# Autodesk Inventor assembly: Сборка1
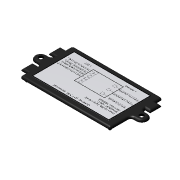
[picture p0: Inventor's stored thumbnail of the model, 180x180]
Saved by Autodesk Inventor 2012 (Build 160160000, 160)
## iProperties
Created: 2009-10-05
Part Number: Сборка1
Document SubType Name: Assembly
Designer: toma
Mass: 4.81656 g
Surface Area: 92.9962 cm^2
Volume: 4.81656 cm^3
Density: 1 g/cm^3
Author: toma
## Documents named in this file (3)
- D:\VSS_WORK\VSS_ENERGO\Сумматор light\КД\Сумматор Light\Сборка1.iam
- D:\VSS_WORK\VSS_ENERGO\Сумматор light\КД\Сумматор Light\крышка.ipt
- D:\VSS_WORK\VSS_ENERGO\Сумматор light\КД\Сумматор Light\наклейка.ipt
## Components (2 placed, 2 different names)
1. крышка:1 — Совмещение:1, Совмещение:2, Совмещение:3
2. наклейка:1 — Совмещение:1, Совмещение:2, Совмещение:3
## Relationships (3: Mate 3)
- Совмещение:1 [Mate]: крышка:1 ↔ наклейка:1
- Совмещение:2 [Mate] (3.5 mm): крышка:1 ↔ наклейка:1
- Совмещение:3 [Mate] (2.5 mm): крышка:1 ↔ наклейка:1
